# Autodesk Inventor assembly: non integrated hatch
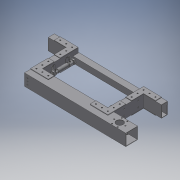
[picture p0: Inventor's stored thumbnail of the model, 180x180]
Saved by Autodesk Inventor 2018 (Build 220112000, 112)
## iProperties
Created: 2019-01-26
Part Number: non integrated hatch
Document SubType Name: Assembly
Designer: s-4008082
Author: s-4008082
## Documents named in this file (7)
- C:\Users\s-4008082\Downloads\2019CAD-master\2019CAD-master\new Hatch design but everythig is broke\non integrated hatch.iam
- C:\Users\s-4008082\Downloads\2019CAD-master\2019CAD-master\new Hatch design but everythig is broke\left arm.ipt
- C:\Users\s-4008082\Downloads\2019CAD-master\2019CAD-master\new Hatch design but everythig is broke\push bar.ipt
- C:\Users\s-4008082\Downloads\2019CAD-master\2019CAD-master\new Hatch design but everythig is broke\PARTserver02019011803125824465437192d056f\AIS2018\021-DXP(F,D-770).iam
- C:\Users\s-4008082\Downloads\2019CAD-master\2019CAD-master\new Hatch design but everythig is broke\Bracing 3x3.ipt
- C:\Users\s-4008082\Downloads\2019CAD-master\2019CAD-master\new Hatch design but everythig is broke\ATACHMENT BAR.ipt
- C:\Users\s-4008082\Downloads\2019CAD-master\2019CAD-master\new Hatch design but everythig is broke\bar thing.ipt
## Components (16 placed, 6 different names)
1. left arm:1 — Flush:23, Flush:34, Mate:41, Mate:42, Flush:37, Mate:47, Mate:51, Mate:55, Mate:59, Mate:60, Flush:50, Flush:51, Mate:67, Mate:68
2. push bar:1
3. 021-DXP(F,D-770):1 [sub-assembly] — Mate:41, Mate:42, Flush:37, Mate:47, Flush:43, Flush:46, Flush:47
4. 021-DXP(F,D-770):2 [sub-assembly] — Flush:43, Mate:50, Flush:46, Flush:47
5. ATACHMENT BAR:1 — Mate:51, Flush:48, Flush:49, Mate:52, Mate:54, Mate:56, Mate:57, Mate:61, Mate:62, Mate:64, Mate:65
6. bar thing:1 — Flush:23, Flush:34, Mate:58, Mate:66, Flush:51
7. bar thing:2 — Flush:52, Flush:53, Mate:71, Mate:72, Mate:75
8. left arm:2 — Mate:50, Flush:48, Flush:49, Mate:53, Mate:63, Mate:70, Flush:52, Flush:53, Mate:71, Mate:73, Mate:74, Mate:76
9. Bracing 3x3:1 — Flush:50, Mate:64, Mate:65
10. Bracing 3x3:2 — Mate:66, Mate:67, Mate:68
11. Bracing 3x3:3 — Mate:70, Mate:72, Mate:73
12. Bracing 3x3:4 — Mate:61, Mate:62, Mate:63
13. Bracing 3x3:5 — Mate:74, Mate:75, Mate:76
14. Bracing 3x3:6 — Mate:58, Mate:59, Mate:60
15. Bracing 3x3:7 — Mate:55, Mate:56, Mate:57
16. Bracing 3x3:8 — Mate:52, Mate:53, Mate:54
## Relationships (45: Mate 33, Flush 12)
- [Mate] (2.54 mm): push bar:1 ↔ 021-DXP(F,D-770):2
- [Mate]: push bar:1 ↔ 021-DXP(F,D-770):2
- [Mate] (2.54 mm): push bar:1 ↔ 021-DXP(F,D-770):1
- [Mate]: push bar:1 ↔ 021-DXP(F,D-770):1
- Flush:23: left arm:1 ↔ bar thing:1
- Flush:34: left arm:1 ↔ bar thing:1
- Mate:41: left arm:1 ↔ 021-DXP(F,D-770):1
- Mate:42: left arm:1 ↔ 021-DXP(F,D-770):1
- Flush:37 (38.1 mm): left arm:1 ↔ 021-DXP(F,D-770):1
- Mate:47: left arm:1 ↔ 021-DXP(F,D-770):1
- Flush:43: 021-DXP(F,D-770):1 ↔ 021-DXP(F,D-770):2
- Mate:50: 021-DXP(F,D-770):2 ↔ left arm:2
- Flush:46: 021-DXP(F,D-770):1 ↔ 021-DXP(F,D-770):2
- Flush:47: 021-DXP(F,D-770):1 ↔ 021-DXP(F,D-770):2
- Mate:51: left arm:1 ↔ ATACHMENT BAR:1
- Flush:48: ATACHMENT BAR:1 ↔ left arm:2
- Flush:49: ATACHMENT BAR:1 ↔ left arm:2
- Mate:52: ATACHMENT BAR:1 ↔ Bracing 3x3:8
- Mate:53: left arm:2 ↔ Bracing 3x3:8
- Mate:54: ATACHMENT BAR:1 ↔ Bracing 3x3:8
- Mate:55: left arm:1 ↔ Bracing 3x3:7
- Mate:56: ATACHMENT BAR:1 ↔ Bracing 3x3:7
- Mate:57: ATACHMENT BAR:1 ↔ Bracing 3x3:7
- Mate:58: bar thing:1 ↔ Bracing 3x3:6
- Mate:59: left arm:1 ↔ Bracing 3x3:6
- Mate:60: left arm:1 ↔ Bracing 3x3:6
- Mate:61: ATACHMENT BAR:1 ↔ Bracing 3x3:4
- Mate:62: ATACHMENT BAR:1 ↔ Bracing 3x3:4
- Mate:63: left arm:2 ↔ Bracing 3x3:4
- Flush:50: left arm:1 ↔ Bracing 3x3:1
- Mate:64: ATACHMENT BAR:1 ↔ Bracing 3x3:1
- Mate:65: ATACHMENT BAR:1 ↔ Bracing 3x3:1
- Mate:66: bar thing:1 ↔ Bracing 3x3:2
- Flush:51: left arm:1 ↔ bar thing:1
- Mate:67: left arm:1 ↔ Bracing 3x3:2
- Mate:68: left arm:1 ↔ Bracing 3x3:2
- Mate:70: left arm:2 ↔ Bracing 3x3:3
- Flush:52: bar thing:2 ↔ left arm:2
- Flush:53: bar thing:2 ↔ left arm:2
- Mate:71: bar thing:2 ↔ left arm:2
- Mate:72: bar thing:2 ↔ Bracing 3x3:3
- Mate:73: left arm:2 ↔ Bracing 3x3:3
- Mate:74: left arm:2 ↔ Bracing 3x3:5
- Mate:75: bar thing:2 ↔ Bracing 3x3:5
- Mate:76: left arm:2 ↔ Bracing 3x3:5
